# Autodesk Inventor assembly: QHY183-Jobin-Yvon
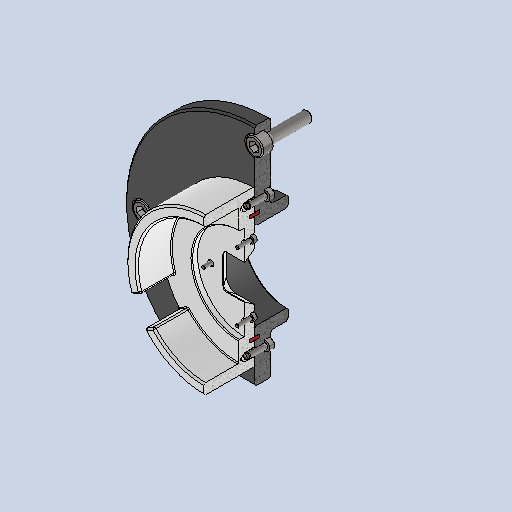
[picture p0: Inventor's stored thumbnail of the model, 512x512]
Saved by Autodesk Inventor 2026 (Build 300175050, 175E)
## iProperties
Created: 2025-02-17
Part Number: QHY183-Jobin-Yvon
Document SubType Name: Assembly
Designer: kuzmin
Author: kuzmin
## Documents named in this file (8)
- C:\Users\queez\Dropbox\Drawings\PIHTI\Jobin-Yvon\QHY183-Jobin-Yvon.iam
- C:\Users\queez\Dropbox\Drawings\PIHTI\Jobin-Yvon\QHY183-flange-adapter.ipt
- C:\Users\queez\Dropbox\Drawings\PIHTI\Jobin-Yvon\Jobin-Yvon-mounting-plate.ipt
- C:\Users\queez\Dropbox\Drawings\PIHTI\ContentCenter\Fastners\M6x25-SHCS.ipt
- C:\Users\queez\Dropbox\Drawings\PIHTI\ContentCenter\Fastners\M3x10-SHCS.ipt
- C:\Users\queez\Dropbox\Drawings\PIHTI\ContentCenter\Fastners\brass-insert-m3x5.ipt
- C:\Users\queez\Dropbox\Drawings\PIHTI\ContentCenter\Fastners\M2x8-SHCS.ipt
- C:\Users\queez\Dropbox\Drawings\PIHTI\Jobin-Yvon\light-seam.ipt
## Components (18 placed, 7 different names)
1. QHY183-flange-adapter:1 — Rigid:1, Rigid:6, Rigid:7, Rigid:8, Rigid:9, Rigid:17, Rigid:18, Rigid:19, Rigid:20
2. Jobin-Yvon-mounting-plate:1 — Rigid:1, Rigid:2, Rigid:3, Rigid:4, Rigid:5, Rigid:14, Rigid:15, Rigid:16, Rotational:1
3. brass-insert-m3x5:1 — Rigid:7
4. brass-insert-m3x5:2 — Rigid:6
5. brass-insert-m3x5:3 — Rigid:8
6. brass-insert-m3x5:4 — Rigid:9
7. light-seam:1 — Rotational:1
8. SS ISO 4762 M2 x 8:1 — Rigid:19
9. SS ISO 4762 M2 x 8:2 — Rigid:17
10. SS ISO 4762 M2 x 8:3 — Rigid:18
11. SS ISO 4762 M2 x 8:4 — Rigid:20
12. IS 2269 M6 x 25:1 — Rigid:15
13. IS 2269 M6 x 25:2 — Rigid:14
14. IS 2269 M6 x 25:3 — Rigid:16
15. JIS B 1176 - Metric M3 x 10:1 — Rigid:4
16. JIS B 1176 - Metric M3 x 10:2 — Rigid:5
17. JIS B 1176 - Metric M3 x 10:3 — Rigid:3
18. JIS B 1176 - Metric M3 x 10:4 — Rigid:2
## Relationships (17: WeldJoint 16, RevoluteJoint 1)
- Rigid:1 [WeldJoint]: QHY183-flange-adapter:1 ↔ Jobin-Yvon-mounting-plate:1
- Rigid:2 [WeldJoint]: Jobin-Yvon-mounting-plate:1 ↔ JIS B 1176 - Metric M3 x 10:4
- Rigid:3 [WeldJoint]: Jobin-Yvon-mounting-plate:1 ↔ JIS B 1176 - Metric M3 x 10:3
- Rigid:4 [WeldJoint]: Jobin-Yvon-mounting-plate:1 ↔ JIS B 1176 - Metric M3 x 10:1
- Rigid:5 [WeldJoint]: Jobin-Yvon-mounting-plate:1 ↔ JIS B 1176 - Metric M3 x 10:2
- Rigid:6 [WeldJoint]: QHY183-flange-adapter:1 ↔ brass-insert-m3x5:2
- Rigid:7 [WeldJoint]: QHY183-flange-adapter:1 ↔ brass-insert-m3x5:1
- Rigid:8 [WeldJoint]: QHY183-flange-adapter:1 ↔ brass-insert-m3x5:3
- Rigid:9 [WeldJoint]: QHY183-flange-adapter:1 ↔ brass-insert-m3x5:4
- Rigid:14 [WeldJoint]: Jobin-Yvon-mounting-plate:1 ↔ IS 2269 M6 x 25:2
- Rigid:15 [WeldJoint]: Jobin-Yvon-mounting-plate:1 ↔ IS 2269 M6 x 25:1
- Rigid:16 [WeldJoint]: Jobin-Yvon-mounting-plate:1 ↔ IS 2269 M6 x 25:3
- Rigid:17 [WeldJoint]: QHY183-flange-adapter:1 ↔ SS ISO 4762 M2 x 8:2
- Rigid:18 [WeldJoint]: QHY183-flange-adapter:1 ↔ SS ISO 4762 M2 x 8:3
- Rigid:19 [WeldJoint]: QHY183-flange-adapter:1 ↔ SS ISO 4762 M2 x 8:1
- Rigid:20 [WeldJoint]: QHY183-flange-adapter:1 ↔ SS ISO 4762 M2 x 8:4
- Rotational:1 [RevoluteJoint]: Jobin-Yvon-mounting-plate:1 ↔ light-seam:1
